# Autodesk Inventor assembly: Cover Assembly v3
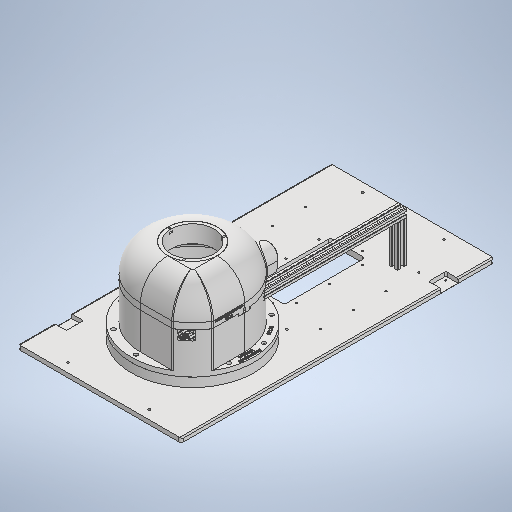
[picture p0: Inventor's stored thumbnail of the model, 512x512]
Saved by Autodesk Inventor 2025 (Build 290162000, 162)
## iProperties
Created: 2025-09-05
Part Number: Cover Assembly v3
Document SubType Name: Assembly
Designer: mumin
Author: mumin
## Documents named in this file (10)
- C:\GitHub\In-situ-monitoring-of-powder-bed-fusion-additive-manufacturing\system_development\Orichalcum\v0.3\Cover Assembly v3.iam
- C:\GitHub\In-situ-monitoring-of-powder-bed-fusion-additive-manufacturing\system_development\Orichalcum\v0.3\Cover v3 Assembly\12mm Cover_orc_v3.ipt
- C:\GitHub\In-situ-monitoring-of-powder-bed-fusion-additive-manufacturing\system_development\Orichalcum\v0.3\Cover v3 Assembly\SealedGlassRing.ipt
- C:\GitHub\In-situ-monitoring-of-powder-bed-fusion-additive-manufacturing\system_development\Orichalcum\v0.3\Cylinder Housing_base_2.ipt
- C:\GitHub\In-situ-monitoring-of-powder-bed-fusion-additive-manufacturing\system_development\Orichalcum\v0.3\Cover v3 Assembly\2020 LV-GVS Beam (530).ipt
- C:\GitHub\In-situ-monitoring-of-powder-bed-fusion-additive-manufacturing\system_development\Orichalcum\v0.3\Cover v3 Assembly\2020 Legs (90mm).ipt
- C:\GitHub\In-situ-monitoring-of-powder-bed-fusion-additive-manufacturing\system_development\Orichalcum\v0.3\Cylinder Housing_cap_2.ipt
- C:\GitHub\In-situ-monitoring-of-powder-bed-fusion-additive-manufacturing\system_development\Orichalcum\v0.3\CenterCylinder_2.ipt
- C:\GitHub\In-situ-monitoring-of-powder-bed-fusion-additive-manufacturing\system_development\Orichalcum\v0.2\Hardware_design\galvo-scanner\GVS_.Mount.ipt
- C:\GitHub\In-situ-monitoring-of-powder-bed-fusion-additive-manufacturing\system_development\Orichalcum\v0.2\Hardware_design\galvo-scanner\GVS102-Step.ipt
## Components (9 placed, 9 different names)
1. 12mm Cover_orc_v3:1 — Insert:1, Insert:10
2. SealedGlassRing:1 — Insert:1, Insert:5, Insert:6
3. 2020 LV-GVS Beam (530):1 — Mate:2, Mate:3, Flush:4
4. Cylinder Housing_base_2:1 — Insert:5, Insert:6, Insert:7
5. Cylinder Housing_cap_2:1 — Insert:7, Insert:8
6. CenterCylinder_2:1 — Insert:8
7. GVS_.Mount:1 — Mate:2, Mate:3, Insert:9, Flush:3
8. GVS102-Step:1 — Insert:9, Flush:3
9. 2020 Legs (90mm):1 — Insert:10, Flush:4
## Relationships (11: Insert 7, Mate 2, Flush 2)
- Insert:1: 12mm Cover_orc_v3:1 ↔ SealedGlassRing:1
- Insert:5: SealedGlassRing:1 ↔ Cylinder Housing_base_2:1
- Insert:6: SealedGlassRing:1 ↔ Cylinder Housing_base_2:1
- Insert:7: Cylinder Housing_base_2:1 ↔ Cylinder Housing_cap_2:1
- Insert:8: Cylinder Housing_cap_2:1 ↔ CenterCylinder_2:1
- Mate:2: 2020 LV-GVS Beam (530):1 ↔ GVS_.Mount:1
- Mate:3: 2020 LV-GVS Beam (530):1 ↔ GVS_.Mount:1
- Insert:9: GVS_.Mount:1 ↔ GVS102-Step:1
- Flush:3: GVS_.Mount:1 ↔ GVS102-Step:1
- Insert:10: 12mm Cover_orc_v3:1 ↔ 2020 Legs (90mm):1
- Flush:4: 2020 LV-GVS Beam (530):1 ↔ 2020 Legs (90mm):1
